# Autodesk Inventor assembly: Assembly1
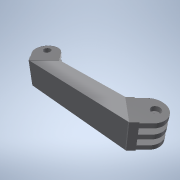
[picture p0: Inventor's stored thumbnail of the model, 180x180]
Saved by Autodesk Inventor 2020 (Build 240168000, 168)
## iProperties
Created: 2020-11-08
Part Number: Assembly1
Document SubType Name: Assembly
Designer: user
Author: user
## Documents named in this file (3)
- C:\Users\user\Downloads\Raspberry_Pi_Camera_Mount_for_MP_Select_Mini\files\Imported Components\Joint_-_only_for_test\Assembly1.iam
- C:\Users\user\Downloads\Raspberry_Pi_Camera_Mount_for_MP_Select_Mini\files\Imported Components\Joint_-_only_for_test\Joint_-_only_for_test.ipt
- C:\Users\user\Downloads\Raspberry_Pi_Camera_Mount_for_MP_Select_Mini\files\Imported Components\Joint_-_only_for_test\Middle.ipt
## Components (3 placed, 2 different names)
1. Joint_-_only_for_test:1 — Mate:1, Flush:1, Flush:4, Symmetry:1, Mate:4
2. Middle:1 — Mate:1, Flush:1, Mate:2, Flush:2, Flush:3, Angle:1, Mate:3, Mate:4
3. Joint_-_only_for_test:2 — Mate:2, Flush:2, Flush:3, Angle:1, Flush:4, Symmetry:1, Mate:3
## Relationships (10: Mate 4, Flush 4, Angle 1, Symmetry 1)
- Mate:1: Joint_-_only_for_test:1 ↔ Middle:1
- Flush:1: Joint_-_only_for_test:1 ↔ Middle:1
- Mate:2: Middle:1 ↔ Joint_-_only_for_test:2
- Flush:2: Middle:1 ↔ Joint_-_only_for_test:2
- Flush:3: Middle:1 ↔ Joint_-_only_for_test:2
- Angle:1 (45 deg): Middle:1 ↔ Joint_-_only_for_test:2
- Flush:4: Joint_-_only_for_test:1 ↔ Joint_-_only_for_test:2
- Symmetry:1: Joint_-_only_for_test:1 ↔ Joint_-_only_for_test:2
- Mate:3: Middle:1 ↔ Joint_-_only_for_test:2
- Mate:4: Joint_-_only_for_test:1 ↔ Middle:1
